# Autodesk Inventor assembly: Baugruppe2
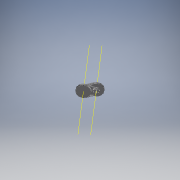
[picture p0: Inventor's stored thumbnail of the model, 180x180]
Saved by Autodesk Inventor 2018.3 (Build 223284000, 284)
## iProperties
Created: 2018-07-27
Part Number: Baugruppe2
Material: Generisch
Document SubType Name: Assembly
Designer: JochenAlt
Author: JochenAlt
## Documents named in this file (3)
- D:\Projects\FlowerPot\CAD\Beltdrive\BeltDriveConstruction.iam
- D:\Projects\FlowerPot\CAD\Beltdrive\Konstruktions-Assistent\Übertragung des Zahnriemens1.iam
- D:\Projects\FlowerPot\CAD\Beltdrive\BeltDriveConstruction\Konstruktions-Assistent\Übertragung des Zahnriemens2.iam
## Components (2 placed, 1 different names)
1. Übertragung des Zahnriemens:3 [sub-assembly] — Passend:8, Passend:14, Passend:15, Passend:16, Drehung:1, Passend:17, Passend:18, Passend:19, Passend:20
2. Übertragung des Zahnriemens:5 [sub-assembly] — Passend:15, Passend:16, Drehung:1, Passend:17, Passend:18, Passend:19, Passend:20
## Relationships (9: Mate 8, RelateRotation 1)
- Passend:8 [Mate]: Übertragung des Zahnriemens:3
- Passend:14 [Mate]: Übertragung des Zahnriemens:3
- Passend:15 [Mate]: Übertragung des Zahnriemens:3 ↔ Übertragung des Zahnriemens:5
- Passend:16 [Mate]: Übertragung des Zahnriemens:3 ↔ Übertragung des Zahnriemens:5
- Drehung:1 [RelateRotation] (-0.48 ul): Übertragung des Zahnriemens:3 ↔ Übertragung des Zahnriemens:5
- Passend:17 [Mate]: Übertragung des Zahnriemens:3 ↔ Übertragung des Zahnriemens:5
- Passend:18 [Mate] (1 mm): Übertragung des Zahnriemens:3 ↔ Übertragung des Zahnriemens:5
- Passend:19 [Mate]: Übertragung des Zahnriemens:3 ↔ Übertragung des Zahnriemens:5
- Passend:20 [Mate]: Übertragung des Zahnriemens:3 ↔ Übertragung des Zahnriemens:5
